# Autodesk Inventor assembly: Static Gantry Assembly
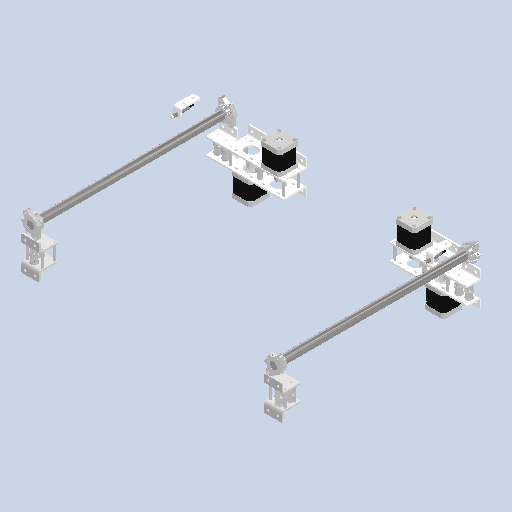
[picture p0: Inventor's stored thumbnail of the model, 512x512]
Saved by Autodesk Inventor 2024 (Build 280153000, 153)
## iProperties
Created: 2024-12-28
Part Number: Static Gantry Assembly
Document SubType Name: Assembly
Designer: Ishaan
Author: Ishaan
## Documents named in this file (11)
- E:\Projects\Axiom--IDEX-3D-Printer\CAD\04 - Gantry\Static Gantry Assembly.iam
- E:\Projects\Axiom--IDEX-3D-Printer\CAD\04 - Gantry\16mm Linear Shaft.ipt
- E:\Projects\Axiom--IDEX-3D-Printer\CAD\00 - COTS Components\SHF16\SHF16.ipt
- E:\Projects\Axiom--IDEX-3D-Printer\CAD\Rev V Envelope Frame Study.ipt
- E:\Projects\Axiom--IDEX-3D-Printer\CAD\04 - Gantry\Left Idler Assembly.iam
- E:\Projects\Axiom--IDEX-3D-Printer\CAD\04 - Gantry\Left XY Drive Mount.iam
- E:\Projects\Axiom--IDEX-3D-Printer\CAD\04 - Gantry\Right Idler Assembly.iam
- E:\Projects\Axiom--IDEX-3D-Printer\CAD\04 - Gantry\Right XY Drive Mount.iam
- E:\Projects\Axiom--IDEX-3D-Printer\CAD\04 - Gantry\Gantry Assembly.iam
- E:\Projects\Axiom--IDEX-3D-Printer\CAD\04 - Gantry\Inductive Sensor Bracket.ipt
- E:\Projects\Axiom--IDEX-3D-Printer\CAD\00 - COTS Components\6mm Inductive Probe\6mm Inductive Probe.ipt
## Components (16 placed, 10 different names)
1. Rev V Envelope Frame Study:1 — Mate:1, Mate:2, Mate:3, Mate:4, Mate:5, Mate:6, Flush:1, Mate:7, Mate:8, Mate:9, Mate:10, Mate:11, Mate:20, Mate:21, Flush:11, Mate:22, Flush:12
2. 16mm Linear Shaft:1 — Insert:1, Insert:2, Mate:4, Mate:12, Mate:15, Mate:16
3. SHF16:1 — Insert:2, Mate:1, Mate:3, Angle:1
4. SHF16:2 — Insert:1, Mate:2, Angle:1
5. 16mm Linear Shaft:2 — Insert:4, Mate:7, Mate:13, Mate:14, Mate:17
6. SHF16:3 — Insert:4, Mate:5, Flush:1
7. SHF16:4 — Mate:6
8. Left Idler Assembly:1 [sub-assembly] — Mate:11, Flush:2, Mate:17
9. Left XY Drive Mount:1 [sub-assembly] — Mate:8, Flush:2, Flush:3, Flush:5, Mate:14
10. Right Idler Assembly:1 [sub-assembly] — Mate:10, Mate:16, Mate:19, Flush:15
11. Right XY Drive Mount:1 [sub-assembly] — Mate:9, Flush:3, Mate:15, Mate:18, Flush:15
12. Gantry Assembly:1 [sub-assembly] — Mate:12, Mate:13, Flush:5, Flush:6, Flush:7, Flush:9, Mate:18, Mate:19
13. Inductive Sensor Bracket:1 — Mate:20, Mate:21, Insert:5, Flush:13
14. Inductive Sensor Bracket:2 — Mate:22, Flush:12, Flush:13, Mate:23
15. 6mm Inductive Probe:1 — Insert:5, Flush:11, Flush:14
16. 6mm Inductive Probe:2 — Mate:23, Flush:14
## Relationships (44: Mate 23, Flush 14, Insert 5, Angle 2)
- Insert:1 (-1 mm): 16mm Linear Shaft:1 ↔ SHF16:2
- Insert:2 (-1 mm): 16mm Linear Shaft:1 ↔ SHF16:1
- Mate:1: Rev V Envelope Frame Study:1 ↔ SHF16:1
- Mate:2: Rev V Envelope Frame Study:1 ↔ SHF16:2
- Mate:3 (-20 mm): Rev V Envelope Frame Study:1 ↔ SHF16:1
- Angle:1 (180 deg): SHF16:1 ↔ SHF16:2
- Mate:4 (50 mm): Rev V Envelope Frame Study:1 ↔ 16mm Linear Shaft:1
- [Insert] (-1 mm): 16mm Linear Shaft:2 ↔ SHF16:4
- Insert:4 (-1 mm): 16mm Linear Shaft:2 ↔ SHF16:3
- [Angle] (180 deg): SHF16:3 ↔ SHF16:4
- Mate:5: Rev V Envelope Frame Study:1 ↔ SHF16:3
- Mate:6: Rev V Envelope Frame Study:1 ↔ SHF16:4
- Flush:1 (20 mm): Rev V Envelope Frame Study:1 ↔ SHF16:3
- Mate:7 (50 mm): Rev V Envelope Frame Study:1 ↔ 16mm Linear Shaft:2
- Mate:8: Rev V Envelope Frame Study:1 ↔ Left XY Drive Mount:1
- Mate:9: Rev V Envelope Frame Study:1 ↔ Right XY Drive Mount:1
- Mate:10: Rev V Envelope Frame Study:1 ↔ Right Idler Assembly:1
- Mate:11: Rev V Envelope Frame Study:1 ↔ Left Idler Assembly:1
- Flush:2: Left Idler Assembly:1 ↔ Left XY Drive Mount:1
- Flush:3: Left XY Drive Mount:1 ↔ Right XY Drive Mount:1
- Mate:12: 16mm Linear Shaft:1 ↔ Gantry Assembly:1
- Mate:13: 16mm Linear Shaft:2 ↔ Gantry Assembly:1
- Flush:5: Left XY Drive Mount:1 ↔ Gantry Assembly:1
- Mate:14: 16mm Linear Shaft:2 ↔ Left XY Drive Mount:1
- Mate:15: 16mm Linear Shaft:1 ↔ Right XY Drive Mount:1
- Mate:16: 16mm Linear Shaft:1 ↔ Right Idler Assembly:1
- Mate:17: 16mm Linear Shaft:2 ↔ Left Idler Assembly:1
- Flush:6 (10 mm): Gantry Assembly:1
- Flush:7 (41 mm): Gantry Assembly:1
- Flush:8 (250 mm)
- Flush:9 (-33 mm): Gantry Assembly:1
- Flush:10 (-25 mm)
- Mate:18 (2 mm): Right XY Drive Mount:1 ↔ Gantry Assembly:1
- Mate:19 (2 mm): Right Idler Assembly:1 ↔ Gantry Assembly:1
- Mate:20 (-10 mm): Rev V Envelope Frame Study:1 ↔ Inductive Sensor Bracket:1
- Mate:21: Rev V Envelope Frame Study:1 ↔ Inductive Sensor Bracket:1
- Insert:5 (-8 mm): Inductive Sensor Bracket:1 ↔ 6mm Inductive Probe:1
- Flush:11 (-109.5 mm): Rev V Envelope Frame Study:1 ↔ 6mm Inductive Probe:1
- Mate:22: Rev V Envelope Frame Study:1 ↔ Inductive Sensor Bracket:2
- Flush:12 (10 mm): Rev V Envelope Frame Study:1 ↔ Inductive Sensor Bracket:2
- Flush:13: Inductive Sensor Bracket:1 ↔ Inductive Sensor Bracket:2
- Mate:23: Inductive Sensor Bracket:2 ↔ 6mm Inductive Probe:2
- Flush:14: 6mm Inductive Probe:1 ↔ 6mm Inductive Probe:2
- Flush:15: Right Idler Assembly:1 ↔ Right XY Drive Mount:1
## Named parameters: d13_d6 = -1 mm, d14_d7 = -1 mm, d15_d11 = 180 deg
